# Autodesk Inventor assembly: ABD_Slider_Set
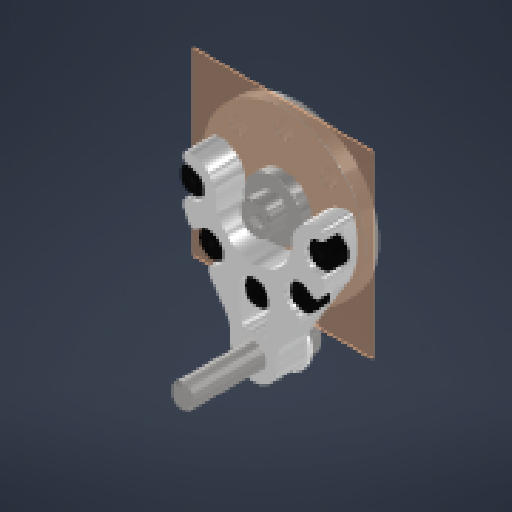
[picture p0: Inventor's stored thumbnail of the model, 512x512]
Saved by Autodesk Inventor 2024.3 (Build 283343000, 343)
## iProperties
Created: 2024-02-15
Part Number: ABD_Slider_Set
Document SubType Name: Assembly
Designer: ASUS
Author: ASUS
## Documents named in this file (7)
- C:\Users\ASUS\Desktop\Anti_Backlash_Structure_OP\V2_Frame(2025)\ABD_Slider_Set_v2.iam
- C:\Users\ASUS\Desktop\2024_Robit_Hardware\ROBOCUP_2024_eindhoven\부품\ROBOTIS(Inventor 2023 ver.)\혼\64-106Horn.ipt
- C:\Users\ASUS\Desktop\Anti_Backlash_Structure_OP\MISUMI\CSH-STN-M3-10_203.ipt
- C:\Users\ASUS\Desktop\Anti_Backlash_Structure_OP\MISUMI\4mm_ABD_set.iam
- C:\Users\ASUS\Desktop\Anti_Backlash_Structure_OP\V2_Frame(2025)\CSHBTT-ST-M4-18_203.ipt
- C:\Users\ASUS\Desktop\Anti_Backlash_Structure_OP\MISUMI\TT-0409-051.ipt
- C:\Users\ASUS\Desktop\Anti_Backlash_Structure_OP\v2_Frame\Slider_crank_horn_v2.ipt
## Components (6 placed, 6 different names)
1. 64-106Horn:1 — 삽입:3, 삽입:11, 메이트:2
2. CSH-STN-M3-10_203:1 — 삽입:3
3. 4mm_ABD_set:1 [sub-assembly] — 삽입:10, 메이트:1, 메이트:2
4. TT-0409-051:1 — 삽입:9, 삽입:12
5. CSHBTT-ST-M4-18_203:1 — 삽입:9
6. Slider_crank_horn_v2:1 — 삽입:10, 메이트:1, 삽입:11, 삽입:12
## Relationships (7: Insert 5, Mate 2)
- 삽입:3 [Insert]: 64-106Horn:1 ↔ CSH-STN-M3-10_203:1
- 삽입:9 [Insert]: TT-0409-051:1 ↔ CSHBTT-ST-M4-18_203:1
- 삽입:10 [Insert]: 4mm_ABD_set:1 ↔ Slider_crank_horn_v2:1
- 메이트:1 [Mate]: 4mm_ABD_set:1 ↔ Slider_crank_horn_v2:1
- 삽입:11 [Insert]: 64-106Horn:1 ↔ Slider_crank_horn_v2:1
- 메이트:2 [Mate]: 64-106Horn:1 ↔ 4mm_ABD_set:1
- 삽입:12 [Insert]: TT-0409-051:1 ↔ Slider_crank_horn_v2:1
